# Autodesk Inventor assembly: Micro_Mate-N-Lok_TE-Connectivity_3mm_1x4_Female
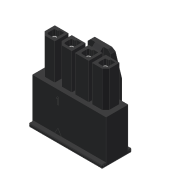
[picture p0: Inventor's stored thumbnail of the model, 180x180]
Saved by Autodesk Inventor 2015 (Build 190159000, 159)
## iProperties
Created: 2015-01-30
Part Number: Micro_Mate-N-Lok_TE-Connectivity_3mm_1x4_Female
Document SubType Name: Assembly
## Documents named in this file (3)
- C:\Dropbox\Inventor\Projects\001_EK-Teile\Micro_Mate-N-Lok_TE-Connectivity_3mm_1x4_Female.iam
- C:\Dropbox\Inventor\Projects\001_EK-Teile\Micro_Mate-N-Lok_TE-Connectivity_3mm_1x4_Female_1445022-4.ipt
- C:\Dropbox\Inventor\Projects\001_EK-Teile\Micro_Mate-N-Lok_TE-Connectivity_3mm_Crimp-Contact_794610-1.ipt
## Components (5 placed, 2 different names)
1. Micro_Mate-N-Lok_TE-Connectivity_3mm_1x4_Female_1445022-4:1 — Mate:1, Mate:2, Flush:1
2. Micro_Mate-N-Lok_TE-Connectivity_3mm_Crimp-Contact_794610-1:1 — Mate:1, Mate:2, Flush:1
3. Micro_Mate-N-Lok_TE-Connectivity_3mm_Crimp-Contact_794610-1:2
4. Micro_Mate-N-Lok_TE-Connectivity_3mm_Crimp-Contact_794610-1:3
5. Micro_Mate-N-Lok_TE-Connectivity_3mm_Crimp-Contact_794610-1:4
## Component patterns: (4 elements, first: Micro_Mate-N-Lok_TE-Connectivity_3mm_Crimp-Contact_794610-1:1)
## Relationships (3: Mate 2, Flush 1)
- Mate:1 (0.062 mm): Micro_Mate-N-Lok_TE-Connectivity_3mm_1x4_Female_1445022-4:1 ↔ Micro_Mate-N-Lok_TE-Connectivity_3mm_Crimp-Contact_794610-1:1
- Mate:2 (0.045 mm): Micro_Mate-N-Lok_TE-Connectivity_3mm_1x4_Female_1445022-4:1 ↔ Micro_Mate-N-Lok_TE-Connectivity_3mm_Crimp-Contact_794610-1:1
- Flush:1 (-0.1 mm): Micro_Mate-N-Lok_TE-Connectivity_3mm_1x4_Female_1445022-4:1 ↔ Micro_Mate-N-Lok_TE-Connectivity_3mm_Crimp-Contact_794610-1:1
